# Autodesk Inventor assembly: mx28_withHorn
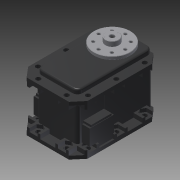
[picture p0: Inventor's stored thumbnail of the model, 180x180]
Saved by Autodesk Inventor 2016 (Build 200138000, 138)
## iProperties
Created: 2014-04-23
Part Number: mx28_withHorn
Document SubType Name: Assembly
Designer: BitBots
Mass: 44.0409 g
Surface Area: 119.943 cm^2
Volume: 44.0409 cm^3
Density: 1 g/cm^3
Author: BitBots
## Documents named in this file (3)
- Z:\NICU\NICO_CAD_master\motors\Mx28\mx28_with_horn.iam
- Z:\NICU\NICO_CAD_master\motors\Mx28\RX-28.ipt
- Z:\NICU\NICO_CAD_master\motors\HN07-N101_(mx28)\HN07-N101.ipt
## Components (2 placed, 2 different names)
1. RX-28:1 — Rotational:2
2. HN07-N101:1 — Rotational:2
## Relationships (1: RevoluteJoint 1)
- Rotational:2 [RevoluteJoint]: RX-28:1 ↔ HN07-N101:1
